# Autodesk Inventor assembly: Assembly1
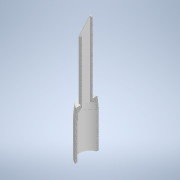
[picture p0: Inventor's stored thumbnail of the model, 180x180]
Saved by Autodesk Inventor 2020.2 (Build 242310000, 310)
## iProperties
Created: 2020-09-23
Part Number: Assembly1
Document SubType Name: Assembly
Designer: Amaan Khalid
Author: Amaan Khalid
## Documents named in this file (3)
- C:\Users\Amaan Khalid\Desktop\My projects\Vaccum Atachment\Assembly1.iam
- C:\Users\Amaan Khalid\Desktop\My projects\Vaccum Atachment\cylinder part.ipt
- C:\Users\Amaan Khalid\Desktop\My projects\Vaccum Atachment\nozzle.ipt
## Components (2 placed, 2 different names)
1. cylinder part:1 — Mate:1
2. nozzle:1 — Mate:1
## Relationships (1: Mate 1)
- Mate:1: cylinder part:1 ↔ nozzle:1
